# Autodesk Inventor assembly: ASY GBK предварительная торцевая
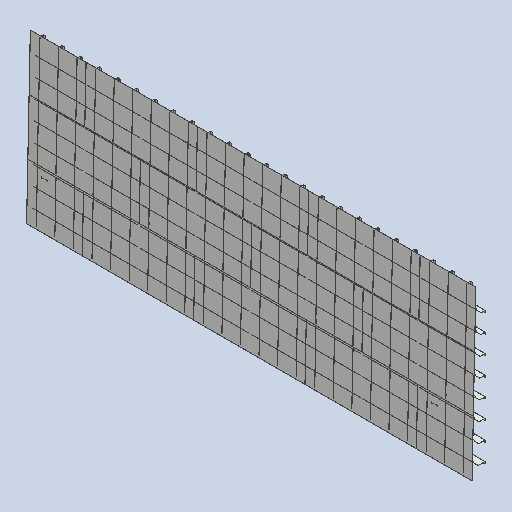
[picture p0: Inventor's stored thumbnail of the model, 512x512]
Saved by Autodesk Inventor 2026 (Build 300175000, 175)
## iProperties
Created: 2026-05-20
Part Number: ASY GBK предварительная торцевая
Document SubType Name: Assembly
Designer: admin
Mass: 2.96106e+06 g
Surface Area: 1.91261e+06 cm^2
Volume: 377205 cm^3
Density: 7.85 g/cm^3
Author: admin
## Documents named in this file (6)
- C:\Users\pokla\Documents\Inventor\GBK-Gubkinskiy\ASY GBK предварительная торцевая.iam
- C:\Users\pokla\Documents\Inventor\GBK-Gubkinskiy\ASY GBK 1110 long wall shield 1.iam
- C:\Users\pokla\Documents\Inventor\GBK-Gubkinskiy\ASY GBK 1120 long wall shield 2.iam
- C:\Users\pokla\Documents\Inventor\GBK-Gubkinskiy\ASY GBK 1210 long wall shield 3.iam
- C:\Users\pokla\Documents\Inventor\GBK-Gubkinskiy\ASY GBK 1310 long wall shield 4.iam
- C:\Users\pokla\Documents\Inventor\GBK-Gubkinskiy\ASY GBK 1320 long wall shield 5.iam
## Components (14 placed, 5 different names)
1. ASY GBK 1110 long wall shield 1.iam:1 [sub-assembly]
2. ASY GBK 1120 long wall shield 2.iam:1 [sub-assembly]
3. ASY GBK 1210 long wall shield 3.iam:1 [sub-assembly]
4. ASY GBK 1310 long wall shield 4.iam:1 [sub-assembly]
5. ASY GBK 1320 long wall shield 5.iam:1 [sub-assembly]
6. ASY GBK 1320 long wall shield 5.iam:2 [sub-assembly]
7. ASY GBK 1320 long wall shield 5.iam:3 [sub-assembly]
8. ASY GBK 1210 long wall shield 3.iam:2 [sub-assembly]
9. ASY GBK 1210 long wall shield 3.iam:3 [sub-assembly]
10. ASY GBK 1210 long wall shield 3.iam:4 [sub-assembly]
11. ASY GBK 1120 long wall shield 2.iam:2 [sub-assembly]
12. ASY GBK 1120 long wall shield 2.iam:3 [sub-assembly]
13. ASY GBK 1310 long wall shield 4.iam:2 [sub-assembly]
14. ASY GBK 1110 long wall shield 1.iam:2 [sub-assembly]
## Relationships (13: WeldJoint 13)
- [WeldJoint] (1 mm): ASY GBK 1110 long wall shield 1.iam:1 ↔ ASY GBK 1120 long wall shield 2.iam:1
- [WeldJoint]: ASY GBK 1110 long wall shield 1.iam:1 ↔ ASY GBK 1210 long wall shield 3.iam:1
- [WeldJoint]: ASY GBK 1210 long wall shield 3.iam:1 ↔ ASY GBK 1310 long wall shield 4.iam:1
- [WeldJoint] (1 mm): ASY GBK 1310 long wall shield 4.iam:1 ↔ ASY GBK 1320 long wall shield 5.iam:1
- [WeldJoint] (1 mm): ASY GBK 1320 long wall shield 5.iam:1 ↔ ASY GBK 1320 long wall shield 5.iam:2
- [WeldJoint] (1 mm): ASY GBK 1320 long wall shield 5.iam:2 ↔ ASY GBK 1320 long wall shield 5.iam:3
- [WeldJoint] (1 mm): ASY GBK 1210 long wall shield 3.iam:1 ↔ ASY GBK 1210 long wall shield 3.iam:2
- [WeldJoint] (1 mm): ASY GBK 1210 long wall shield 3.iam:2 ↔ ASY GBK 1210 long wall shield 3.iam:3
- [WeldJoint] (1 mm): ASY GBK 1210 long wall shield 3.iam:3 ↔ ASY GBK 1210 long wall shield 3.iam:4
- [WeldJoint] (1 mm): ASY GBK 1120 long wall shield 2.iam:1 ↔ ASY GBK 1120 long wall shield 2.iam:2
- [WeldJoint] (1 mm): ASY GBK 1120 long wall shield 2.iam:2 ↔ ASY GBK 1120 long wall shield 2.iam:3
- [WeldJoint] (1 mm): ASY GBK 1320 long wall shield 5.iam:3 ↔ ASY GBK 1310 long wall shield 4.iam:2
- [WeldJoint] (1 mm): ASY GBK 1120 long wall shield 2.iam:3 ↔ ASY GBK 1110 long wall shield 1.iam:2
## Named parameters: d141_Зазор_по_горизонту = 1 mm, d142_d99 = 0 mm, d152_d98 = 0 mm
